# Autodesk Inventor assembly: IMU_housing
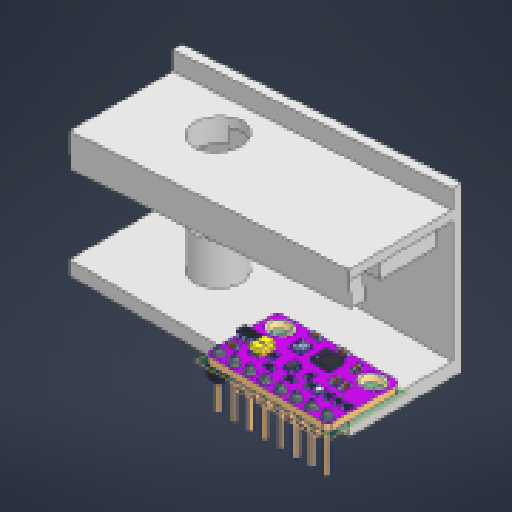
[picture p0: Inventor's stored thumbnail of the model, 512x512]
Saved by Autodesk Inventor 2026.1 (Build 301233020, 233B)
## iProperties
Created: 2025-12-04
Part Number: IMU_housing
Document SubType Name: Assembly
Designer: jaewook
Author: jaewook
## Documents named in this file (4)
- C:\Users\kjh19\Documents\Inventor\project\turrte_projict_v2\IMU_housing.iam
- C:\Users\kjh19\Documents\Inventor\project\turrte_projict_v2\GY-91_MPU9250+BMP280 - Pins Down.ipt
- C:\Users\kjh19\Documents\Inventor\project\turrte_projict_v2\IMU_base.ipt
- C:\Users\kjh19\Documents\Inventor\project\turrte_projict_v2\part2.ipt
## Components (3 placed, 3 different names)
1. GY-91_MPU9250+BMP280 - Pins Down:1 — 플러쉬:1
2. IMU_base:1 — 플러쉬:1, 플러쉬:2, 플러쉬:3
3. part2:1 — 플러쉬:2, 플러쉬:3
## Relationships (3: Flush 3)
- 플러쉬:1 [Flush]: GY-91_MPU9250+BMP280 - Pins Down:1 ↔ IMU_base:1
- 플러쉬:2 [Flush]: IMU_base:1 ↔ part2:1
- 플러쉬:3 [Flush]: IMU_base:1 ↔ part2:1
